# Autodesk Inventor assembly: Gantry
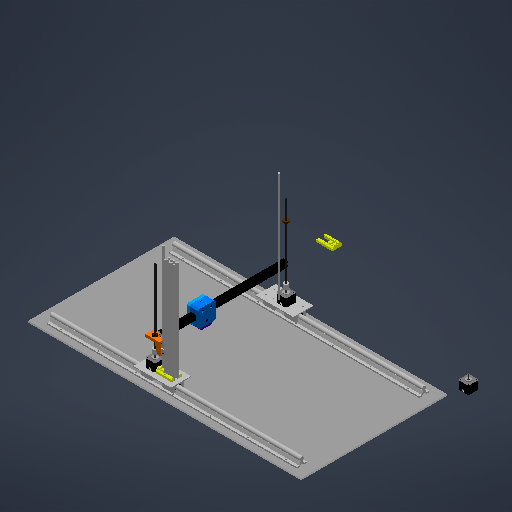
[picture p0: Inventor's stored thumbnail of the model, 512x512]
Saved by Autodesk Inventor 2025.1 (Build 291241000, 241)
## iProperties
Created: 2024-10-31
Part Number: Gantry
Document SubType Name: Assembly
Designer: jerem
Author: jerem
## Documents named in this file (16)
- C:\Users\jerem\Documents\GitHub\Perovskite-Automated-Synthesis-System\CAD\Complete System.iam
- C:\Users\jerem\Documents\GitHub\Perovskite-Automated-Synthesis-System\CAD\Non 3D Printed Parts\Base Plate.ipt
- C:\Users\jerem\Documents\GitHub\Perovskite-Automated-Synthesis-System\CAD\Non 3D Printed Parts\Linear Rails\Linear Rail.ipt
- C:\Users\jerem\Documents\GitHub\Perovskite-Automated-Synthesis-System\CAD\Non 3D Printed Parts\Linear Rails\Linear Rail Slider Block.ipt
- C:\Users\jerem\Documents\GitHub\Perovskite-Automated-Synthesis-System\CAD\Camera\Camera Assembly.iam
- C:\Users\jerem\Documents\GitHub\Perovskite-Automated-Synthesis-System\CAD\Toolhead\Toolhead.iam
- C:\Users\jerem\Documents\GitHub\Perovskite-Automated-Synthesis-System\CAD\Non 3D Printed Parts\X Axis Base Plate.ipt
- C:\Users\jerem\Documents\GitHub\Perovskite-Automated-Synthesis-System\CAD\Non 3D Printed Parts\Extrusion\V Extrustion 40x400mm.ipt
- C:\Users\jerem\Documents\GitHub\Perovskite-Automated-Synthesis-System\CAD\Non 3D Printed Parts\Extrusion\V Extrustion 20x500mm.ipt
- C:\Users\jerem\Documents\GitHub\Perovskite-Automated-Synthesis-System\CAD\Non 3D Printed Parts\Motors and Servos\NEMA17 Stepper Motor.ipt
- C:\Users\jerem\Documents\GitHub\Perovskite-Automated-Synthesis-System\CAD\Non 3D Printed Parts\Threaded Rod 300mm.ipt
- C:\Users\jerem\Documents\GitHub\Perovskite-Automated-Synthesis-System\CAD\Non 3D Printed Parts\Rod Coupler.ipt
- C:\Users\jerem\Documents\GitHub\Perovskite-Automated-Synthesis-System\CAD\Non 3D Printed Parts\Leadscrew.ipt
- C:\Users\jerem\Documents\GitHub\Perovskite-Automated-Synthesis-System\CAD\Gantry\Rot Bottom Mount.ipt
- C:\Users\jerem\Documents\GitHub\Perovskite-Automated-Synthesis-System\CAD\Non 3D Printed Parts\Linear Rails\8mm Linear Rod.ipt
- C:\Users\jerem\Documents\GitHub\Perovskite-Automated-Synthesis-System\CAD\Gantry\Z-Y Axis Bracket.iam
## Components (26 placed, 15 different names)
1. Base Plate:1 — Flush:1, Flush:2, Mate:1, Mate:2, Angle:1, Angle:2, Angle:3, Angle:4, Angle:5, Angle:8
2. Linear Rail:1 — Flush:1, Flush:2, Mate:1, Flush:3, Mate:3, Mate:4, Mate:5
3. Linear Rail:2 — Mate:2, Flush:3, Mate:3, Mate:6, Mate:7
4. Linear Rail Slider Block:1 — Mate:4, Angle:4, Mate:21, Mate:22, Mate:51
5. Linear Rail Slider Block:2 — Mate:5, Angle:3, Flush:5, Mate:20
6. Linear Rail Slider Block:3 — Mate:6, Angle:1, Flush:5, Mate:26, Mate:27
7. Linear Rail Slider Block:4 — Mate:7, Angle:2, Mate:25
8. Camera Assembly:1 [sub-assembly] — Mate:17, Mate:18, Mate:19
9. Toolhead:1 [sub-assembly] — Mate:17, Angle:5, Mate:18, Mate:19, Mate:28, Mate:29
10. X Axis Base Plate:1 — Mate:20, Mate:21, Mate:22, Mate:23, Angle:6, Mate:31, Mate:42, Mate:44
11. X Axis Base Plate:2 — Mate:25, Mate:26, Mate:27, Mate:30
12. V Extrustion 40x400mm:1 — Mate:23, Angle:6, Mate:49, Mate:50
13. V Extrustion 20x500mm:1 — Angle:8, Mate:28, Mate:29, Mate:52
14. NEMA17 Stepper Motor:1 — Mate:31, Mate:32, Mate:38, Mate:45
15. NEMA17 Stepper Motor:2 — Mate:30, Mate:33, Mate:36
16. Threaded Rod 300mm:1 — Mate:34, Mate:39, Mate:47
17. Rod Coupler:1 — Mate:32, Mate:34, Mate:38, Mate:39
18. Rod Coupler:2 — Mate:33, Mate:35, Mate:36, Mate:37
19. Threaded Rod 300mm:2 — Mate:35, Mate:37, Mate:41
20. Leadscrew:2 — Mate:41
21. Rot Bottom Mount:1
22. Rot Bottom Mount:2 — Mate:42, Mate:43, Mate:45, Mate:49, Mate:50, Mate:51
23. 8mm Linear Rod:1 — Mate:43, Mate:44, Mate:48
24. 8mm Linear Rod:2
25. Z-Y Axis Bracket:1 [sub-assembly] — Mate:47, Mate:48, Mate:52
26. NEMA17 Stepper Motor:3
## Relationships (51: Mate 40, Angle 7, Flush 4)
- Flush:1 (50 mm): Base Plate:1 ↔ Linear Rail:1
- Flush:2 (25 mm): Base Plate:1 ↔ Linear Rail:1
- Mate:1: Base Plate:1 ↔ Linear Rail:1
- Mate:2: Base Plate:1 ↔ Linear Rail:2
- Flush:3: Linear Rail:1 ↔ Linear Rail:2
- Mate:3 (450 mm): Linear Rail:1 ↔ Linear Rail:2
- Mate:4: Linear Rail:1 ↔ Linear Rail Slider Block:1
- Mate:5: Linear Rail:1 ↔ Linear Rail Slider Block:2
- Mate:6: Linear Rail:2 ↔ Linear Rail Slider Block:3
- Mate:7: Linear Rail:2 ↔ Linear Rail Slider Block:4
- Angle:1 (0 deg): Base Plate:1 ↔ Linear Rail Slider Block:3
- Angle:2 (0 deg): Base Plate:1 ↔ Linear Rail Slider Block:4
- Angle:3 (0 deg): Base Plate:1 ↔ Linear Rail Slider Block:2
- Angle:4 (0 deg): Base Plate:1 ↔ Linear Rail Slider Block:1
- Flush:5: Linear Rail Slider Block:2 ↔ Linear Rail Slider Block:3
- Mate:17: Camera Assembly:1 ↔ Toolhead:1
- Angle:5 (0 deg): Base Plate:1 ↔ Toolhead:1
- Mate:18: Camera Assembly:1 ↔ Toolhead:1
- Mate:19: Camera Assembly:1 ↔ Toolhead:1
- Mate:20: Linear Rail Slider Block:2 ↔ X Axis Base Plate:1
- Mate:21: Linear Rail Slider Block:1 ↔ X Axis Base Plate:1
- Mate:22: Linear Rail Slider Block:1 ↔ X Axis Base Plate:1
- Mate:23: X Axis Base Plate:1 ↔ V Extrustion 40x400mm:1
- Angle:6 (0 deg): X Axis Base Plate:1 ↔ V Extrustion 40x400mm:1
- Mate:25: Linear Rail Slider Block:4 ↔ X Axis Base Plate:2
- Mate:26: Linear Rail Slider Block:3 ↔ X Axis Base Plate:2
- Mate:27: Linear Rail Slider Block:3 ↔ X Axis Base Plate:2
- Angle:8 (0 deg): Base Plate:1 ↔ V Extrustion 20x500mm:1
- Mate:28: Toolhead:1 ↔ V Extrustion 20x500mm:1
- Mate:29: Toolhead:1 ↔ V Extrustion 20x500mm:1
- Mate:30: X Axis Base Plate:2 ↔ NEMA17 Stepper Motor:2
- Mate:31: X Axis Base Plate:1 ↔ NEMA17 Stepper Motor:1
- Mate:32: NEMA17 Stepper Motor:1 ↔ Rod Coupler:1
- Mate:33: NEMA17 Stepper Motor:2 ↔ Rod Coupler:2
- Mate:34: Threaded Rod 300mm:1 ↔ Rod Coupler:1
- Mate:35: Rod Coupler:2 ↔ Threaded Rod 300mm:2
- Mate:36 (-8 mm): NEMA17 Stepper Motor:2 ↔ Rod Coupler:2
- Mate:37 (-8 mm): Rod Coupler:2 ↔ Threaded Rod 300mm:2
- Mate:38 (-8 mm): NEMA17 Stepper Motor:1 ↔ Rod Coupler:1
- Mate:39 (-8 mm): Threaded Rod 300mm:1 ↔ Rod Coupler:1
- Mate:41: Threaded Rod 300mm:2 ↔ Leadscrew:2
- Mate:42: X Axis Base Plate:1 ↔ Rot Bottom Mount:2
- Mate:43: Rot Bottom Mount:2 ↔ 8mm Linear Rod:1
- Mate:44: X Axis Base Plate:1 ↔ 8mm Linear Rod:1
- Mate:45: NEMA17 Stepper Motor:1 ↔ Rot Bottom Mount:2
- Mate:47: Threaded Rod 300mm:1 ↔ Z-Y Axis Bracket:1
- Mate:48: 8mm Linear Rod:1 ↔ Z-Y Axis Bracket:1
- Mate:49: V Extrustion 40x400mm:1 ↔ Rot Bottom Mount:2
- Mate:50: V Extrustion 40x400mm:1 ↔ Rot Bottom Mount:2
- Mate:51: Linear Rail Slider Block:1 ↔ Rot Bottom Mount:2
- Mate:52: V Extrustion 20x500mm:1 ↔ Z-Y Axis Bracket:1
